# Autodesk Inventor assembly: 齿轮箱1
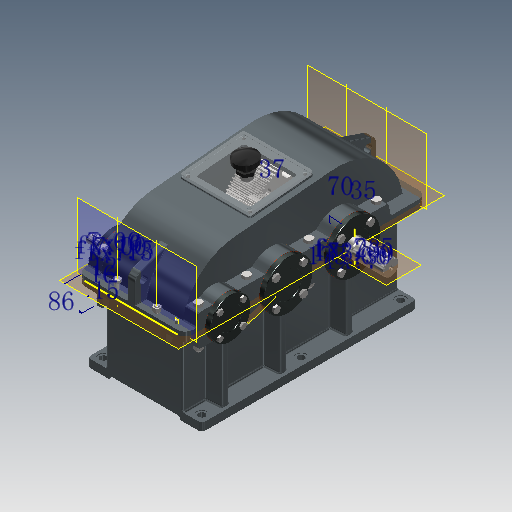
[picture p0: Inventor's stored thumbnail of the model, 512x512]
Saved by Autodesk Inventor 2025 (Build 290162000, 162)
## iProperties
Created: 2025-03-10
Part Number: 齿轮箱1
Document SubType Name: Assembly
Designer: liukan
Author: liukan
## Documents named in this file (40)
- D:\2025春夏那些过往\2025春夏课程文件\机械设计课程设计（甲）\Inventor files\齿轮箱.iam
- D:\2025春夏那些过往\2025春夏课程文件\机械设计课程设计（甲）\Inventor files\下半箱体.ipt
- D:\2025春夏那些过往\2025春夏课程文件\机械设计课程设计（甲）\Inventor files\高速轴.iam
- D:\2025春夏那些过往\2025春夏课程文件\机械设计课程设计（甲）\Inventor files\中间轴.iam
- D:\2025春夏那些过往\2025春夏课程文件\机械设计课程设计（甲）\Inventor files\低速轴.iam
- D:\2025春夏那些过往\2025春夏课程文件\机械设计课程设计（甲）\Inventor files\高速齿轮.iam
- D:\2025春夏那些过往\2025春夏课程文件\机械设计课程设计（甲）\Inventor files\低速齿轮.iam
- D:\2025春夏那些过往\2025春夏课程文件\机械设计课程设计（甲）\Inventor files\齿轮箱\设计加速器\键联接1.iam
- D:\2025春夏那些过往\2025春夏课程文件\机械设计课程设计（甲）\Inventor files\齿轮箱\设计加速器\键联接2.iam
- D:\2025春夏那些过往\2025春夏课程文件\机械设计课程设计（甲）\Inventor files\齿轮箱\设计加速器\键联接3.iam
- D:\2025春夏那些过往\2025春夏课程文件\机械设计课程设计（甲）\Inventor files\齿轮箱\设计加速器\键联接4.iam
- D:\2025春夏那些过往\2025春夏课程文件\机械设计课程设计（甲）\Inventor files\上半箱体.ipt
- D:\2025春夏那些过往\2025春夏课程文件\机械设计课程设计（甲）\Inventor files\轴承盖\轴承盖1无孔.ipt
- D:\2025春夏那些过往\2025春夏课程文件\机械设计课程设计（甲）\Inventor files\轴承盖\轴承盖1有孔.ipt
- D:\2025春夏那些过往\2025春夏课程文件\机械设计课程设计（甲）\Inventor files\轴承盖\轴承盖2.ipt
- D:\2025春夏那些过往\2025春夏课程文件\机械设计课程设计（甲）\Inventor files\轴承盖\轴承盖3无孔.ipt
- D:\2025春夏那些过往\2025春夏课程文件\机械设计课程设计（甲）\Inventor files\轴承盖\轴承盖3有孔.ipt
- D:\2025春夏那些过往\2025春夏课程文件\机械设计课程设计（甲）\Inventor files\调整垫片\调整垫片1.ipt
- D:\2025春夏那些过往\2025春夏课程文件\机械设计课程设计（甲）\Inventor files\调整垫片\调整垫片2.ipt
- D:\2025春夏那些过往\2025春夏课程文件\机械设计课程设计（甲）\Inventor files\调整垫片\调整垫片3.ipt
- D:\2025春夏那些过往\2025春夏课程文件\机械设计课程设计（甲）\Inventor files\杆式油标.ipt
- D:\2025春夏那些过往\2025春夏课程文件\机械设计课程设计（甲）\Inventor files\排油孔\封油垫.ipt
- D:\2025春夏那些过往\2025春夏课程文件\机械设计课程设计（甲）\Inventor files\排油孔\排油孔螺塞.ipt
- D:\2025春夏那些过往\2025春夏课程文件\机械设计课程设计（甲）\Inventor files\检查孔\盖板.ipt
- D:\2025春夏那些过往\2025春夏课程文件\机械设计课程设计（甲）\Inventor files\检查孔\滤网.ipt
- D:\2025春夏那些过往\2025春夏课程文件\机械设计课程设计（甲）\Inventor files\检查孔\通气器盖子.ipt
- D:\2025春夏那些过往\2025春夏课程文件\机械设计课程设计（甲）\Inventor files\检查孔\通气器主体.ipt
- D:\2025春夏那些过往\2025春夏课程文件\机械设计课程设计（甲）\Inventor files\定位销.ipt
- D:\文档\Inventor\Content Center Files\R2025\zh-CN\GB_T 5783-2000\螺栓 GB_T 5783 M10 x 25.ipt
- D:\文档\Inventor\Content Center Files\R2025\zh-CN\GB_T 5782-2000\螺栓 GB_T 5782 M10 x 35.ipt
- D:\文档\Inventor\Content Center Files\R2025\zh-CN\GB_T 5782-2000\螺栓 GB_T 5782 M12 x 100.ipt
- D:\文档\Inventor\Content Center Files\R2025\zh-CN\GB_T 6170-2000\螺母 GB_T 6170 M10.ipt
- D:\文档\Inventor\Content Center Files\R2025\zh-CN\GB_T 6170-2000\螺母 GB_T 6170 M12.ipt
- D:\文档\Inventor\Content Center Files\R2025\zh-CN\GB 93-87\垫圈 GB 93-87 10.ipt
- D:\文档\Inventor\Content Center Files\R2025\zh-CN\GB 93-87\垫圈 GB 93-87 12.ipt
- D:\文档\Inventor\Content Center Files\R2025\zh-CN\GB_T 5783-2000\螺栓 GB_T 5783 M8 x 25.ipt
- D:\2025春夏那些过往\2025春夏课程文件\机械设计课程设计（甲）\Inventor files\轴承盖\高速轴油封.ipt
- D:\2025春夏那些过往\2025春夏课程文件\机械设计课程设计（甲）\Inventor files\轴承盖\低速轴油封.ipt
- D:\2025春夏那些过往\2025春夏课程文件\机械设计课程设计（甲）\Inventor files\中间轴\中间轴套筒.ipt
- D:\2025春夏那些过往\2025春夏课程文件\机械设计课程设计（甲）\Inventor files\低速轴\低速轴套筒.ipt
## Components (95 placed, 38 different names)
1. 下半箱体:1 — 表面齐平:1, 表面齐平:2, 表面齐平:3, 角度:1, 表面齐平:4, 配合:15, 表面齐平:12, 表面齐平:13, 配合:21, 配合:23, 配合:25, 配合:27, 配合:29, 配合:31, 配合:36, 配合:40, 配合:42, 配合:44, 配合:54, 配合:55, 配合:56, 配合:57, 配合:58, 表面齐平:25, 表面齐平:30, 配合:69, 配合:77, 配合:78, 配合:81, 配合:90, 配合:94, 配合:118, 配合:123, 配合:124, 配合:129, 配合:130, 配合:135, 配合:136, 配合:140, 配合:141, 配合:240, 配合:241, 配合:242, 配合:243, 配合:244, 配合:245, 配合:246, 配合:247
2. 上半箱体:1 — 表面齐平:12, 表面齐平:13, 配合:34, 配合:38, 配合:65, 配合:66, 配合:67, 表面齐平:23, 配合:68, 表面齐平:26, 表面齐平:27, 表面齐平:29, 配合:70, 配合:79, 配合:80, 配合:89, 配合:91, 配合:92, 配合:93, 配合:117, 配合:121, 配合:122, 配合:126, 配合:127, 配合:128, 配合:133, 配合:134
3. 高速轴:1 [sub-assembly] — 角度:1, 配合:2, 配合:231
4. 中间轴:1 [sub-assembly] — 角度:2, 配合:1, 配合:5, 配合:6, 角度:9, 配合:8, 角度:11, 配合:15, 表面齐平:40, 配合:225, 配合:232, 表面齐平:47, 角度:55, 配合:248, 表面齐平:48, 角度:56, 配合:249
5. 低速轴:1 [sub-assembly] — 角度:3, 配合:4, 角度:7, 表面齐平:4, 配合:6, 角度:14, 配合:12, 配合:227, 表面齐平:41, 配合:233, 表面齐平:46, 角度:54, 配合:239, 表面齐平:49, 角度:57, 配合:250
6. 高速齿轮:1 [sub-assembly] — 配合:1, 配合:2, 角度:4, 角度:9, 配合:8, 配合:234
7. 低速齿轮:1 [sub-assembly] — 配合:4, 配合:5, 角度:11, 角度:14, 配合:12, 配合:227
8. 键联接:1 [sub-assembly] — 表面齐平:47, 角度:55, 配合:248
9. 键联接:2 [sub-assembly] — 表面齐平:48, 角度:56, 配合:249
10. 键联接:3 [sub-assembly] — 表面齐平:46, 角度:54, 配合:239
11. 键联接:4 [sub-assembly] — 表面齐平:49, 角度:57, 配合:250
12. 杆式油标:1 — 配合:54, 配合:55
13. 定位销:1 — 表面齐平:23, 配合:68, 表面齐平:24, 表面齐平:25
14. 定位销:2 — 表面齐平:26, 表面齐平:27, 表面齐平:28, 表面齐平:29, 表面齐平:30
15. 起盖螺钉 — 配合:69, 配合:70, 角度:30
16. 中间轴套筒:1 — 表面齐平:40
17. 中间轴套筒:2 — 配合:225, 配合:234
18. 低速轴套筒:1 — 表面齐平:41
19. 高速轴承闷盖 — 配合:21, 配合:22, 角度:21, 配合:43, 配合:45, 配合:146, 配合:147, 配合:152, 配合:153, 配合:154, 配合:155, 配合:156, 配合:157, 配合:158, 配合:159, 配合:160, 配合:161, 配合:231
20. 高速轴承透盖 — 配合:23, 配合:24, 角度:22, 配合:41, 配合:46, 配合:138, 配合:142, 配合:143, 配合:144, 配合:145, 配合:148, 配合:149, 配合:150, 配合:151, 配合:214, 配合:215
21. 高速轴油封:1 — 配合:214, 配合:215
22. 中间轴承闷盖1 — 配合:25, 配合:26, 角度:23, 配合:37, 配合:48, 配合:170, 配合:171, 配合:172, 配合:173, 配合:174, 配合:175, 配合:176, 配合:177, 配合:198, 配合:199, 配合:200, 配合:201, 配合:232
23. 中间轴承闷盖2 — 角度:24, 配合:27, 配合:28, 配合:39, 配合:47, 配合:162, 配合:163, 配合:164, 配合:165, 配合:166, 配合:167, 配合:168, 配合:169, 配合:194, 配合:195, 配合:196, 配合:197
24. 低速轴承闷盖 — 配合:29, 配合:30, 角度:25, 配合:35, 配合:50, 配合:178, 配合:179, 配合:180, 配合:181, 配合:182, 配合:183, 配合:184, 配合:185, 配合:202, 配合:203, 配合:204, 配合:206
25. 低速轴承透盖 — 配合:31, 配合:32, 角度:26, 配合:33, 配合:49, 配合:186, 配合:187, 配合:188, 配合:189, 配合:190, 配合:191, 配合:192, 配合:193, 配合:205, 配合:207, 配合:208, 配合:209, 配合:216, 配合:217, 配合:218, 配合:233
26. 低速轴油封:1 — 配合:216, 配合:217, 配合:218
27. 调整垫片1:1 — 配合:24, 配合:41, 配合:42, 配合:46
28. 调整垫片2:1 — 配合:28, 配合:39, 配合:40, 配合:47
29. 调整垫片3:2 — 配合:32, 配合:33, 配合:34, 配合:49
30. 调整垫片2:2 — 配合:26, 配合:37, 配合:38, 配合:48
31. 调整垫片1:2 — 配合:22, 配合:43, 配合:44, 配合:45
32. 调整垫片3:1 — 配合:30, 配合:35, 配合:36, 配合:50
33. 排油孔螺塞:1 — 配合:58, 配合:59, 配合:137
34. 封油垫片:1 — 配合:56, 配合:57, 配合:59
35. 滤网:1 — 配合:60, 配合:61
36. 通气器盖子:1 — 表面齐平:22, 配合:62
37. 通气器主体:1 — 配合:60, 配合:61, 表面齐平:22, 配合:62, 配合:63, 配合:64
38. 盖板:1 — 配合:63, 配合:64, 配合:65, 配合:66, 配合:67
39. 螺栓 GB/T 5782-2000 M10x35:1 — 配合:74, 配合:75, 配合:77, 配合:78, 角度:31
40. 螺母 GB/T 6170-2000 M10:1 — 配合:74, 配合:76
41. 垫圈 GB/T 93-1987 M10:1 — 配合:75, 配合:76, 配合:79
42. 螺栓 GB/T 5782-2000 M10x35:2 — 配合:91, 配合:90, 角度:32
43. 螺母 GB/T 6170-2000 M10:2
44. 垫圈 GB/T 93-1987 M10:2 — 配合:89
45. 螺栓 GB/T 5782-2000 M10x35:3 — 配合:93, 配合:94
46. 螺母 GB/T 6170-2000 M10:3 — 角度:33
47. 垫圈 GB/T 93-1987 M10:3 — 配合:92
48. 螺母 GB/T 6170-2000 M12:1 — 配合:72, 配合:73
49. 垫圈 GB/T 93-1987 M12:1 — 配合:71, 配合:73, 配合:81
50. 螺栓 GB/T 5782-2000 M12x100:1 — 配合:71, 配合:72, 配合:80, 配合:240
51. 螺栓 GB/T 5782-2000 M12x100:2 — 配合:117, 角度:34, 配合:241
52. 螺母 GB/T 6170-2000 M12:2
53. 垫圈 GB/T 93-1987 M12:2 — 配合:118
54. 螺栓 GB/T 5782-2000 M12x100:3 — 配合:121, 角度:35, 配合:242
55. 螺母 GB/T 6170-2000 M12:3
56. 垫圈 GB/T 93-1987 M12:3 — 配合:124
57. 螺栓 GB/T 5782-2000 M12x100:4 — 配合:122, 角度:36, 配合:243
58. 螺母 GB/T 6170-2000 M12:4
59. 垫圈 GB/T 93-1987 M12:4 — 配合:123
60. 螺栓 GB/T 5782-2000 M12x100:5 — 配合:128, 角度:37, 配合:244
61. 螺母 GB/T 6170-2000 M12:5
62. 垫圈 GB/T 93-1987 M12:5 — 配合:129
63. 螺栓 GB/T 5782-2000 M12x100:6 — 配合:126, 配合:127, 角度:38, 配合:245
64. 螺母 GB/T 6170-2000 M12:6
65. 垫圈 GB/T 93-1987 M12:6 — 配合:130
66. 螺栓 GB/T 5782-2000 M12x100:7 — 配合:134, 角度:39, 配合:246
67. 螺母 GB/T 6170-2000 M12:7
68. 垫圈 GB/T 93-1987 M12:7 — 配合:135
69. 螺栓 GB/T 5782-2000 M12x100:8 — 配合:133, 角度:40, 配合:247
70. 螺母 GB/T 6170-2000 M12:8
71. 垫圈 GB/T 93-1987 M12:8 — 配合:136
72. 螺栓 GB/T 5783-2000 M8 x 25:1 — 配合:143, 配合:148
73. 螺栓 GB/T 5783-2000 M8 x 25:2 — 配合:140, 配合:144, 配合:149
74. 螺栓 GB/T 5783-2000 M8 x 25:3 — 配合:141, 配合:145, 配合:150
75. 螺栓 GB/T 5783-2000 M8 x 25:4 — 配合:138, 配合:142, 配合:151
76. 螺栓 GB/T 5783-2000 M8 x 25:5 — 配合:152, 配合:146, 配合:147
77. 螺栓 GB/T 5783-2000 M8 x 25:6 — 配合:153, 配合:158, 配合:159
78. 螺栓 GB/T 5783-2000 M8 x 25:7 — 配合:154, 配合:157, 配合:160
79. 螺栓 GB/T 5783-2000 M8 x 25:8 — 配合:155, 配合:156, 配合:161
80. 螺栓 GB/T 5783-2000 M10 x 25:2 — 配合:162, 配合:168, 配合:194
81. 螺栓 GB/T 5783-2000 M10 x 25:3 — 配合:163, 配合:169, 配合:195
82. 螺栓 GB/T 5783-2000 M10 x 25:4 — 配合:164, 配合:167, 配合:196
83. 螺栓 GB/T 5783-2000 M10 x 25:5 — 配合:165, 配合:166, 配合:197
84. 螺栓 GB/T 5783-2000 M10 x 25:6 — 配合:170, 配合:171, 配合:198
85. 螺栓 GB/T 5783-2000 M10 x 25:7 — 配合:173, 配合:175, 配合:199
86. 螺栓 GB/T 5783-2000 M10 x 25:8 — 配合:174, 配合:177, 配合:200
87. 螺栓 GB/T 5783-2000 M10 x 25:9 — 配合:172, 配合:176, 配合:201
88. 螺栓 GB/T 5783-2000 M10 x 25:10 — 配合:178, 配合:182, 配合:202
89. 螺栓 GB/T 5783-2000 M10 x 25:11 — 配合:179, 配合:183, 配合:203
90. 螺栓 GB/T 5783-2000 M10 x 25:12 — 配合:180, 配合:184, 配合:204
91. 螺栓 GB/T 5783-2000 M10 x 25:14 — 配合:188, 配合:190, 配合:205
92. 螺栓 GB/T 5783-2000 M10 x 25:13 — 配合:181, 配合:185, 配合:206
93. 螺栓 GB/T 5783-2000 M10 x 25:15 — 配合:189, 配合:193, 配合:207
94. 螺栓 GB/T 5783-2000 M10 x 25:16 — 配合:187, 配合:192, 配合:208
95. 螺栓 GB/T 5783-2000 M10 x 25:17 — 配合:186, 配合:191, 配合:209
## Relationships (259: Mate 209, Angle 29, Flush 21)
- 表面齐平:1 [Flush]: 下半箱体:1
- 表面齐平:2 [Flush]: 下半箱体:1
- 表面齐平:3 [Flush]: 下半箱体:1
- 角度:1 [Angle] (0 deg): 下半箱体:1 ↔ 高速轴:1
- 角度:2 [Angle] (0 deg): 中间轴:1
- 角度:3 [Angle] (0 deg): 低速轴:1
- 配合:1 [Mate]: 中间轴:1 ↔ 高速齿轮:1
- 配合:2 [Mate]: 高速轴:1 ↔ 高速齿轮:1
- 角度:4 [Angle] (180 deg): 高速齿轮:1
- 配合:4 [Mate]: 低速轴:1 ↔ 低速齿轮:1
- 配合:5 [Mate]: 中间轴:1 ↔ 低速齿轮:1
- 角度:7 [Angle] (0 deg): 低速轴:1
- 表面齐平:4 [Flush]: 下半箱体:1 ↔ 低速轴:1
- 配合:6 [Mate]: 中间轴:1 ↔ 低速轴:1
- 角度:9 [Angle] (11.4804 deg): 中间轴:1 ↔ 高速齿轮:1
- 配合:8 [Mate]: 中间轴:1 ↔ 高速齿轮:1
- 角度:11 [Angle] (170.0196 deg): 中间轴:1 ↔ 低速齿轮:1
- 角度:14 [Angle] (88.2353 deg): 低速轴:1 ↔ 低速齿轮:1
- 配合:12 [Mate]: 低速轴:1 ↔ 低速齿轮:1
- 配合:15 [Mate]: 下半箱体:1 ↔ 中间轴:1
- 表面齐平:12 [Flush]: 下半箱体:1 ↔ 上半箱体:1
- 表面齐平:13 [Flush]: 下半箱体:1 ↔ 上半箱体:1
- 配合:21 [Mate]: 下半箱体:1 ↔ 高速轴承闷盖
- 配合:22 [Mate]: 高速轴承闷盖 ↔ 调整垫片1:2
- 角度:21 [Angle] (0 deg): 高速轴承闷盖
- 配合:23 [Mate]: 下半箱体:1 ↔ 高速轴承透盖
- 配合:24 [Mate]: 高速轴承透盖 ↔ 调整垫片1:1
- 角度:22 [Angle] (0 deg): 高速轴承透盖
- 配合:25 [Mate]: 下半箱体:1 ↔ 中间轴承闷盖1
- 配合:26 [Mate]: 中间轴承闷盖1 ↔ 调整垫片2:2
- 角度:23 [Angle] (0 deg): 中间轴承闷盖1
- 角度:24 [Angle] (0 deg): 中间轴承闷盖2
- 配合:27 [Mate]: 下半箱体:1 ↔ 中间轴承闷盖2
- 配合:28 [Mate]: 中间轴承闷盖2 ↔ 调整垫片2:1
- 配合:29 [Mate]: 下半箱体:1 ↔ 低速轴承闷盖
- 配合:30 [Mate]: 低速轴承闷盖 ↔ 调整垫片3:1
- 角度:25 [Angle] (0 deg): 低速轴承闷盖
- 配合:31 [Mate]: 下半箱体:1 ↔ 低速轴承透盖
- 配合:32 [Mate]: 低速轴承透盖 ↔ 调整垫片3:2
- 角度:26 [Angle] (0 deg): 低速轴承透盖
- 配合:33 [Mate]: 低速轴承透盖 ↔ 调整垫片3:2
- 配合:34 [Mate]: 上半箱体:1 ↔ 调整垫片3:2
- 配合:35 [Mate]: 低速轴承闷盖 ↔ 调整垫片3:1
- 配合:36 [Mate]: 下半箱体:1 ↔ 调整垫片3:1
- 配合:37 [Mate]: 中间轴承闷盖1 ↔ 调整垫片2:2
- 配合:38 [Mate]: 上半箱体:1 ↔ 调整垫片2:2
- 配合:39 [Mate]: 中间轴承闷盖2 ↔ 调整垫片2:1
- 配合:40 [Mate]: 下半箱体:1 ↔ 调整垫片2:1
- 配合:41 [Mate]: 高速轴承透盖 ↔ 调整垫片1:1
- 配合:42 [Mate]: 下半箱体:1 ↔ 调整垫片1:1
- 配合:43 [Mate]: 高速轴承闷盖 ↔ 调整垫片1:2
- 配合:44 [Mate]: 下半箱体:1 ↔ 调整垫片1:2
- 配合:45 [Mate]: 高速轴承闷盖 ↔ 调整垫片1:2
- 配合:46 [Mate]: 高速轴承透盖 ↔ 调整垫片1:1
- 配合:47 [Mate]: 中间轴承闷盖2 ↔ 调整垫片2:1
- 配合:48 [Mate]: 中间轴承闷盖1 ↔ 调整垫片2:2
- 配合:49 [Mate]: 低速轴承透盖 ↔ 调整垫片3:2
- 配合:50 [Mate]: 低速轴承闷盖 ↔ 调整垫片3:1
- 配合:54 [Mate]: 下半箱体:1 ↔ 杆式油标:1
- 配合:55 [Mate]: 下半箱体:1 ↔ 杆式油标:1
- 配合:56 [Mate]: 下半箱体:1 ↔ 封油垫片:1
- 配合:57 [Mate]: 下半箱体:1 ↔ 封油垫片:1
- 配合:58 [Mate]: 下半箱体:1 ↔ 排油孔螺塞:1
- 配合:59 [Mate]: 排油孔螺塞:1 ↔ 封油垫片:1
- 配合:60 [Mate]: 滤网:1 ↔ 通气器主体:1
- 配合:61 [Mate]: 滤网:1 ↔ 通气器主体:1
- 表面齐平:22 [Flush]: 通气器盖子:1 ↔ 通气器主体:1
- 配合:62 [Mate]: 通气器盖子:1 ↔ 通气器主体:1
- 配合:63 [Mate]: 通气器主体:1 ↔ 盖板:1
- 配合:64 [Mate]: 通气器主体:1 ↔ 盖板:1
- 配合:65 [Mate]: 上半箱体:1 ↔ 盖板:1
- 配合:66 [Mate]: 上半箱体:1 ↔ 盖板:1
- 配合:67 [Mate]: 上半箱体:1 ↔ 盖板:1
- 表面齐平:23 [Flush]: 上半箱体:1 ↔ 定位销:1
- 配合:68 [Mate]: 上半箱体:1 ↔ 定位销:1
- 表面齐平:24 [Flush] (-100 mm): 定位销:1
- 表面齐平:25 [Flush]: 下半箱体:1 ↔ 定位销:1
- 表面齐平:26 [Flush]: 上半箱体:1 ↔ 定位销:2
- 表面齐平:27 [Flush]: 上半箱体:1 ↔ 定位销:2
- 表面齐平:28 [Flush] (100 mm): 定位销:2
- 表面齐平:29 [Flush]: 上半箱体:1 ↔ 定位销:2
- 表面齐平:30 [Flush]: 下半箱体:1 ↔ 定位销:2
- 配合:69 [Mate]: 下半箱体:1 ↔ 起盖螺钉
- 配合:70 [Mate]: 上半箱体:1 ↔ 起盖螺钉
- 角度:30 [Angle] (0 deg): 起盖螺钉
- 配合:71 [Mate]: 垫圈 GB/T 93-1987 M12:1 ↔ 螺栓 GB/T 5782-2000 M12x100:1
- 配合:72 [Mate]: 螺母 GB/T 6170-2000 M12:1 ↔ 螺栓 GB/T 5782-2000 M12x100:1
- 配合:73 [Mate]: 螺母 GB/T 6170-2000 M12:1 ↔ 垫圈 GB/T 93-1987 M12:1
- 配合:74 [Mate]: 螺栓 GB/T 5782-2000 M10x35:1 ↔ 螺母 GB/T 6170-2000 M10:1
- 配合:75 [Mate]: 螺栓 GB/T 5782-2000 M10x35:1 ↔ 垫圈 GB/T 93-1987 M10:1
- 配合:76 [Mate]: 螺母 GB/T 6170-2000 M10:1 ↔ 垫圈 GB/T 93-1987 M10:1
- 配合:77 [Mate]: 下半箱体:1 ↔ 螺栓 GB/T 5782-2000 M10x35:1
- 配合:78 [Mate]: 下半箱体:1 ↔ 螺栓 GB/T 5782-2000 M10x35:1
- 配合:79 [Mate]: 上半箱体:1 ↔ 垫圈 GB/T 93-1987 M10:1
- 角度:31 [Angle] (0 deg): 螺栓 GB/T 5782-2000 M10x35:1
- 配合:80 [Mate]: 上半箱体:1 ↔ 螺栓 GB/T 5782-2000 M12x100:1
- 配合:81 [Mate]: 下半箱体:1 ↔ 垫圈 GB/T 93-1987 M12:1
- [Mate]: 螺栓 GB/T 5782-2000 M10x35:2 ↔ 螺母 GB/T 6170-2000 M10:2
- [Mate]: 螺栓 GB/T 5782-2000 M10x35:2 ↔ 垫圈 GB/T 93-1987 M10:2
- [Mate]: 螺母 GB/T 6170-2000 M10:2 ↔ 垫圈 GB/T 93-1987 M10:2
- [Mate]: 螺栓 GB/T 5782-2000 M10x35:3 ↔ 螺母 GB/T 6170-2000 M10:3
- [Mate]: 螺栓 GB/T 5782-2000 M10x35:3 ↔ 垫圈 GB/T 93-1987 M10:3
- [Mate]: 螺母 GB/T 6170-2000 M10:3 ↔ 垫圈 GB/T 93-1987 M10:3
- 配合:89 [Mate]: 上半箱体:1 ↔ 垫圈 GB/T 93-1987 M10:2
- 配合:91 [Mate]: 上半箱体:1 ↔ 螺栓 GB/T 5782-2000 M10x35:2
- 配合:90 [Mate]: 下半箱体:1 ↔ 螺栓 GB/T 5782-2000 M10x35:2
- 角度:32 [Angle] (0 deg): 螺栓 GB/T 5782-2000 M10x35:2
- 配合:92 [Mate]: 上半箱体:1 ↔ 垫圈 GB/T 93-1987 M10:3
- 配合:93 [Mate]: 上半箱体:1 ↔ 螺栓 GB/T 5782-2000 M10x35:3
- 配合:94 [Mate]: 下半箱体:1 ↔ 螺栓 GB/T 5782-2000 M10x35:3
- 角度:33 [Angle] (0 deg): 螺母 GB/T 6170-2000 M10:3
- [Mate]: 螺栓 GB/T 5782-2000 M12x100:2 ↔ 垫圈 GB/T 93-1987 M12:2
- [Mate]: 螺栓 GB/T 5782-2000 M12x100:2 ↔ 螺母 GB/T 6170-2000 M12:2
- [Mate]: 螺母 GB/T 6170-2000 M12:2 ↔ 垫圈 GB/T 93-1987 M12:2
- [Mate]: 螺栓 GB/T 5782-2000 M12x100:3 ↔ 垫圈 GB/T 93-1987 M12:3
- [Mate]: 螺栓 GB/T 5782-2000 M12x100:3 ↔ 螺母 GB/T 6170-2000 M12:3
- [Mate]: 螺母 GB/T 6170-2000 M12:3 ↔ 垫圈 GB/T 93-1987 M12:3
- [Mate]: 螺栓 GB/T 5782-2000 M12x100:4 ↔ 垫圈 GB/T 93-1987 M12:4
- [Mate]: 螺栓 GB/T 5782-2000 M12x100:4 ↔ 螺母 GB/T 6170-2000 M12:4
- [Mate]: 螺母 GB/T 6170-2000 M12:4 ↔ 垫圈 GB/T 93-1987 M12:4
- [Mate]: 螺栓 GB/T 5782-2000 M12x100:5 ↔ 垫圈 GB/T 93-1987 M12:5
- [Mate]: 螺栓 GB/T 5782-2000 M12x100:5 ↔ 螺母 GB/T 6170-2000 M12:5
- [Mate]: 螺母 GB/T 6170-2000 M12:5 ↔ 垫圈 GB/T 93-1987 M12:5
- [Mate]: 螺栓 GB/T 5782-2000 M12x100:6 ↔ 垫圈 GB/T 93-1987 M12:6
- [Mate]: 螺栓 GB/T 5782-2000 M12x100:6 ↔ 螺母 GB/T 6170-2000 M12:6
- [Mate]: 螺母 GB/T 6170-2000 M12:6 ↔ 垫圈 GB/T 93-1987 M12:6
- [Mate]: 螺栓 GB/T 5782-2000 M12x100:7 ↔ 垫圈 GB/T 93-1987 M12:7
- [Mate]: 螺栓 GB/T 5782-2000 M12x100:7 ↔ 螺母 GB/T 6170-2000 M12:7
- [Mate]: 螺母 GB/T 6170-2000 M12:7 ↔ 垫圈 GB/T 93-1987 M12:7
- [Mate]: 螺栓 GB/T 5782-2000 M12x100:8 ↔ 垫圈 GB/T 93-1987 M12:8
- [Mate]: 螺栓 GB/T 5782-2000 M12x100:8 ↔ 螺母 GB/T 6170-2000 M12:8
- [Mate]: 螺母 GB/T 6170-2000 M12:8 ↔ 垫圈 GB/T 93-1987 M12:8
- 配合:117 [Mate]: 上半箱体:1 ↔ 螺栓 GB/T 5782-2000 M12x100:2
- 配合:118 [Mate]: 下半箱体:1 ↔ 垫圈 GB/T 93-1987 M12:2
- 配合:121 [Mate]: 上半箱体:1 ↔ 螺栓 GB/T 5782-2000 M12x100:3
- 配合:122 [Mate]: 上半箱体:1 ↔ 螺栓 GB/T 5782-2000 M12x100:4
- 配合:123 [Mate]: 下半箱体:1 ↔ 垫圈 GB/T 93-1987 M12:4
- 配合:124 [Mate]: 下半箱体:1 ↔ 垫圈 GB/T 93-1987 M12:3
- 配合:126 [Mate]: 上半箱体:1 ↔ 螺栓 GB/T 5782-2000 M12x100:6
- 配合:127 [Mate]: 上半箱体:1 ↔ 螺栓 GB/T 5782-2000 M12x100:6
- 配合:128 [Mate]: 上半箱体:1 ↔ 螺栓 GB/T 5782-2000 M12x100:5
- 配合:129 [Mate]: 下半箱体:1 ↔ 垫圈 GB/T 93-1987 M12:5
- 配合:130 [Mate]: 下半箱体:1 ↔ 垫圈 GB/T 93-1987 M12:6
- 配合:133 [Mate]: 上半箱体:1 ↔ 螺栓 GB/T 5782-2000 M12x100:8
- 配合:134 [Mate]: 上半箱体:1 ↔ 螺栓 GB/T 5782-2000 M12x100:7
- 配合:135 [Mate]: 下半箱体:1 ↔ 垫圈 GB/T 93-1987 M12:7
- 配合:136 [Mate]: 下半箱体:1 ↔ 垫圈 GB/T 93-1987 M12:8
- 角度:34 [Angle] (0 deg): 螺栓 GB/T 5782-2000 M12x100:2
- 角度:35 [Angle] (0 deg): 螺栓 GB/T 5782-2000 M12x100:3
- 角度:36 [Angle] (0 deg): 螺栓 GB/T 5782-2000 M12x100:4
- 角度:37 [Angle] (0 deg): 螺栓 GB/T 5782-2000 M12x100:5
- 角度:38 [Angle] (0 deg): 螺栓 GB/T 5782-2000 M12x100:6
- 角度:39 [Angle] (0 deg): 螺栓 GB/T 5782-2000 M12x100:7
- 角度:40 [Angle] (0 deg): 螺栓 GB/T 5782-2000 M12x100:8
- 配合:137 [Mate]: 排油孔螺塞:1
- 配合:138 [Mate]: 高速轴承透盖 ↔ 螺栓 GB/T 5783-2000 M8 x 25:4
- 配合:140 [Mate]: 下半箱体:1 ↔ 螺栓 GB/T 5783-2000 M8 x 25:2
- 配合:141 [Mate]: 下半箱体:1 ↔ 螺栓 GB/T 5783-2000 M8 x 25:3
- 配合:142 [Mate]: 高速轴承透盖 ↔ 螺栓 GB/T 5783-2000 M8 x 25:4
- 配合:143 [Mate]: 高速轴承透盖 ↔ 螺栓 GB/T 5783-2000 M8 x 25:1
- 配合:144 [Mate]: 高速轴承透盖 ↔ 螺栓 GB/T 5783-2000 M8 x 25:2
- 配合:145 [Mate]: 高速轴承透盖 ↔ 螺栓 GB/T 5783-2000 M8 x 25:3
- 配合:149 [Mate]: 高速轴承透盖 ↔ 螺栓 GB/T 5783-2000 M8 x 25:2
- 配合:150 [Mate]: 高速轴承透盖 ↔ 螺栓 GB/T 5783-2000 M8 x 25:3
- 配合:151 [Mate]: 高速轴承透盖 ↔ 螺栓 GB/T 5783-2000 M8 x 25:4
- 配合:152 [Mate]: 高速轴承闷盖 ↔ 螺栓 GB/T 5783-2000 M8 x 25:5
- 配合:146 [Mate]: 高速轴承闷盖 ↔ 螺栓 GB/T 5783-2000 M8 x 25:5
- 配合:147 [Mate]: 高速轴承闷盖 ↔ 螺栓 GB/T 5783-2000 M8 x 25:5
- 配合:148 [Mate]: 高速轴承透盖 ↔ 螺栓 GB/T 5783-2000 M8 x 25:1
- 配合:153 [Mate]: 高速轴承闷盖 ↔ 螺栓 GB/T 5783-2000 M8 x 25:6
- 配合:154 [Mate]: 高速轴承闷盖 ↔ 螺栓 GB/T 5783-2000 M8 x 25:7
- 配合:155 [Mate]: 高速轴承闷盖 ↔ 螺栓 GB/T 5783-2000 M8 x 25:8
- 配合:156 [Mate]: 高速轴承闷盖 ↔ 螺栓 GB/T 5783-2000 M8 x 25:8
- 配合:157 [Mate]: 高速轴承闷盖 ↔ 螺栓 GB/T 5783-2000 M8 x 25:7
- 配合:158 [Mate]: 高速轴承闷盖 ↔ 螺栓 GB/T 5783-2000 M8 x 25:6
- 配合:159 [Mate]: 高速轴承闷盖 ↔ 螺栓 GB/T 5783-2000 M8 x 25:6
- 配合:160 [Mate]: 高速轴承闷盖 ↔ 螺栓 GB/T 5783-2000 M8 x 25:7
- 配合:161 [Mate]: 高速轴承闷盖 ↔ 螺栓 GB/T 5783-2000 M8 x 25:8
- 配合:162 [Mate]: 中间轴承闷盖2 ↔ 螺栓 GB/T 5783-2000 M10 x 25:2
- 配合:163 [Mate]: 中间轴承闷盖2 ↔ 螺栓 GB/T 5783-2000 M10 x 25:3
- 配合:164 [Mate]: 中间轴承闷盖2 ↔ 螺栓 GB/T 5783-2000 M10 x 25:4
- 配合:165 [Mate]: 中间轴承闷盖2 ↔ 螺栓 GB/T 5783-2000 M10 x 25:5
- 配合:166 [Mate]: 中间轴承闷盖2 ↔ 螺栓 GB/T 5783-2000 M10 x 25:5
- 配合:167 [Mate]: 中间轴承闷盖2 ↔ 螺栓 GB/T 5783-2000 M10 x 25:4
- 配合:168 [Mate]: 中间轴承闷盖2 ↔ 螺栓 GB/T 5783-2000 M10 x 25:2
- 配合:169 [Mate]: 中间轴承闷盖2 ↔ 螺栓 GB/T 5783-2000 M10 x 25:3
- 配合:170 [Mate]: 中间轴承闷盖1 ↔ 螺栓 GB/T 5783-2000 M10 x 25:6
- 配合:171 [Mate]: 中间轴承闷盖1 ↔ 螺栓 GB/T 5783-2000 M10 x 25:6
- 配合:172 [Mate]: 中间轴承闷盖1 ↔ 螺栓 GB/T 5783-2000 M10 x 25:9
- 配合:173 [Mate]: 中间轴承闷盖1 ↔ 螺栓 GB/T 5783-2000 M10 x 25:7
- 配合:174 [Mate]: 中间轴承闷盖1 ↔ 螺栓 GB/T 5783-2000 M10 x 25:8
- 配合:175 [Mate]: 中间轴承闷盖1 ↔ 螺栓 GB/T 5783-2000 M10 x 25:7
- 配合:176 [Mate]: 中间轴承闷盖1 ↔ 螺栓 GB/T 5783-2000 M10 x 25:9
- 配合:177 [Mate]: 中间轴承闷盖1 ↔ 螺栓 GB/T 5783-2000 M10 x 25:8
- 配合:178 [Mate]: 低速轴承闷盖 ↔ 螺栓 GB/T 5783-2000 M10 x 25:10
- 配合:179 [Mate]: 低速轴承闷盖 ↔ 螺栓 GB/T 5783-2000 M10 x 25:11
- 配合:180 [Mate]: 低速轴承闷盖 ↔ 螺栓 GB/T 5783-2000 M10 x 25:12
- 配合:181 [Mate]: 低速轴承闷盖 ↔ 螺栓 GB/T 5783-2000 M10 x 25:13
- 配合:182 [Mate]: 低速轴承闷盖 ↔ 螺栓 GB/T 5783-2000 M10 x 25:10
- 配合:183 [Mate]: 低速轴承闷盖 ↔ 螺栓 GB/T 5783-2000 M10 x 25:11
- 配合:184 [Mate]: 低速轴承闷盖 ↔ 螺栓 GB/T 5783-2000 M10 x 25:12
- 配合:185 [Mate]: 低速轴承闷盖 ↔ 螺栓 GB/T 5783-2000 M10 x 25:13
- 配合:186 [Mate]: 低速轴承透盖 ↔ 螺栓 GB/T 5783-2000 M10 x 25:17
- 配合:187 [Mate]: 低速轴承透盖 ↔ 螺栓 GB/T 5783-2000 M10 x 25:16
- 配合:188 [Mate]: 低速轴承透盖 ↔ 螺栓 GB/T 5783-2000 M10 x 25:14
- 配合:189 [Mate]: 低速轴承透盖 ↔ 螺栓 GB/T 5783-2000 M10 x 25:15
- 配合:190 [Mate]: 低速轴承透盖 ↔ 螺栓 GB/T 5783-2000 M10 x 25:14
- 配合:191 [Mate]: 低速轴承透盖 ↔ 螺栓 GB/T 5783-2000 M10 x 25:17
- 配合:192 [Mate]: 低速轴承透盖 ↔ 螺栓 GB/T 5783-2000 M10 x 25:16
- 配合:193 [Mate]: 低速轴承透盖 ↔ 螺栓 GB/T 5783-2000 M10 x 25:15
- 配合:194 [Mate]: 中间轴承闷盖2 ↔ 螺栓 GB/T 5783-2000 M10 x 25:2
- 配合:195 [Mate]: 中间轴承闷盖2 ↔ 螺栓 GB/T 5783-2000 M10 x 25:3
- 配合:196 [Mate]: 中间轴承闷盖2 ↔ 螺栓 GB/T 5783-2000 M10 x 25:4
- 配合:197 [Mate]: 中间轴承闷盖2 ↔ 螺栓 GB/T 5783-2000 M10 x 25:5
- 配合:198 [Mate]: 中间轴承闷盖1 ↔ 螺栓 GB/T 5783-2000 M10 x 25:6
- 配合:199 [Mate]: 中间轴承闷盖1 ↔ 螺栓 GB/T 5783-2000 M10 x 25:7
- 配合:200 [Mate]: 中间轴承闷盖1 ↔ 螺栓 GB/T 5783-2000 M10 x 25:8
- 配合:201 [Mate]: 中间轴承闷盖1 ↔ 螺栓 GB/T 5783-2000 M10 x 25:9
- 配合:202 [Mate]: 低速轴承闷盖 ↔ 螺栓 GB/T 5783-2000 M10 x 25:10
- 配合:203 [Mate]: 低速轴承闷盖 ↔ 螺栓 GB/T 5783-2000 M10 x 25:11
- 配合:204 [Mate]: 低速轴承闷盖 ↔ 螺栓 GB/T 5783-2000 M10 x 25:12
- 配合:205 [Mate]: 低速轴承透盖 ↔ 螺栓 GB/T 5783-2000 M10 x 25:14
- 配合:206 [Mate]: 低速轴承闷盖 ↔ 螺栓 GB/T 5783-2000 M10 x 25:13
- 配合:207 [Mate]: 低速轴承透盖 ↔ 螺栓 GB/T 5783-2000 M10 x 25:15
- 配合:208 [Mate]: 低速轴承透盖 ↔ 螺栓 GB/T 5783-2000 M10 x 25:16
- 配合:209 [Mate]: 低速轴承透盖 ↔ 螺栓 GB/T 5783-2000 M10 x 25:17
- 配合:214 [Mate]: 高速轴承透盖 ↔ 高速轴油封:1
- 配合:215 [Mate]: 高速轴承透盖 ↔ 高速轴油封:1
- 配合:216 [Mate]: 低速轴承透盖 ↔ 低速轴油封:1
- 配合:217 [Mate]: 低速轴承透盖 ↔ 低速轴油封:1
- 配合:218 [Mate]: 低速轴承透盖 ↔ 低速轴油封:1
- 表面齐平:40 [Flush]: 中间轴:1 ↔ 中间轴套筒:1
- 配合:225 [Mate]: 中间轴:1 ↔ 中间轴套筒:2
- 配合:227 [Mate]: 低速轴:1 ↔ 低速齿轮:1
- 表面齐平:41 [Flush]: 低速轴:1 ↔ 低速轴套筒:1
- 配合:231 [Mate]: 高速轴:1 ↔ 高速轴承闷盖
- 配合:232 [Mate]: 中间轴:1 ↔ 中间轴承闷盖1
- 配合:233 [Mate]: 低速轴:1 ↔ 低速轴承透盖
- 配合:234 [Mate]: 高速齿轮:1 ↔ 中间轴套筒:2
- 表面齐平:46 [Flush] (7 mm): 低速轴:1 ↔ 键联接:3
- 角度:54 [Angle] (90 deg): 低速轴:1 ↔ 键联接:3
- 配合:239 [Mate]: 低速轴:1 ↔ 键联接:3
- 配合:240 [Mate]: 下半箱体:1 ↔ 螺栓 GB/T 5782-2000 M12x100:1
- 配合:241 [Mate]: 下半箱体:1 ↔ 螺栓 GB/T 5782-2000 M12x100:2
- 配合:242 [Mate]: 下半箱体:1 ↔ 螺栓 GB/T 5782-2000 M12x100:3
- 配合:243 [Mate]: 下半箱体:1 ↔ 螺栓 GB/T 5782-2000 M12x100:4
- 配合:244 [Mate]: 下半箱体:1 ↔ 螺栓 GB/T 5782-2000 M12x100:5
- 配合:245 [Mate]: 下半箱体:1 ↔ 螺栓 GB/T 5782-2000 M12x100:6
- 配合:246 [Mate]: 下半箱体:1 ↔ 螺栓 GB/T 5782-2000 M12x100:7
- 配合:247 [Mate]: 下半箱体:1 ↔ 螺栓 GB/T 5782-2000 M12x100:8
- 表面齐平:47 [Flush] (6.5 mm): 中间轴:1 ↔ 键联接:1
- 角度:55 [Angle] (189.98 deg): 中间轴:1 ↔ 键联接:1
- 配合:248 [Mate]: 中间轴:1 ↔ 键联接:1
- 表面齐平:48 [Flush] (16.5 mm): 中间轴:1 ↔ 键联接:2
- 角度:56 [Angle] (-9.98 deg): 中间轴:1 ↔ 键联接:2
- 配合:249 [Mate]: 中间轴:1 ↔ 键联接:2
- 表面齐平:49 [Flush] (7.5 mm): 低速轴:1 ↔ 键联接:4
- 角度:57 [Angle] (90 deg): 低速轴:1 ↔ 键联接:4
- 配合:250 [Mate]: 低速轴:1 ↔ 键联接:4
## Named parameters: d170_d153 = 0 mm, d171_d154 = 0 mm, d172_d152 = 0 mm, d173_d170_d153 = 0 mm, d174_d171_d154 = 0 mm, d175_d172_d152 = 0 mm, d196_d151 = 0 mm, d197_d149 = 0 mm, d198_d150 = 0 mm, d199_d151 = 0 mm, d200_d149 = 0 mm, d201_d150 = 0 mm, d202_d151 = 0 mm, d203_d149 = 0 mm, d204_d150 = 0 mm, d205_d151 = 0 mm, d206_d149 = 0 mm, d207_d150 = 0 mm, d208_d151 = 0 mm, d209_d149 = 0 mm, d210_d150 = 0 mm, d211_d151 = 0 mm, d212_d149 = 0 mm, d213_d150 = 0 mm, d214_d151 = 0 mm, d215_d149 = 0 mm, d216_d150 = 0 mm
